# Autodesk Inventor assembly: brama kwadraty
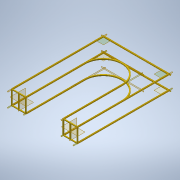
[picture p0: Inventor's stored thumbnail of the model, 180x180]
Saved by Autodesk Inventor 2021 (Build 250183000, 183)
## iProperties
Created: 2024-04-18
Part Number: brama kwadraty
Document SubType Name: Assembly
Designer: Michal
Author: Michal
## Documents named in this file (8)
- C:\Users\Michal\Documents\GitHub\PNW_PhotoBoothFrame_3D\brama kwadraty.iam
- C:\Users\Michal\Documents\GitHub\PNW_PhotoBoothFrame_3D\Lacznik prosty sruby.iam
- C:\Users\Michal\Documents\GitHub\PNW_PhotoBoothFrame_3D\Luk R1000.ipt
- C:\Users\Michal\Documents\GitHub\PNW_PhotoBoothFrame_3D\Stopa v3.iam
- C:\Users\Michal\Documents\GitHub\PNW_PhotoBoothFrame_3D\Naroznik v2.iam
- C:\Users\Michal\Documents\GitHub\PNW_PhotoBoothFrame_3D\Przedluzka L1680.ipt
- C:\Users\Michal\Documents\GitHub\PNW_PhotoBoothFrame_3D\Przedluzka L2400.ipt
- C:\Users\Michal\Documents\GitHub\PNW_PhotoBoothFrame_3D\Przedluzka L1360.ipt
## Components (22 placed, 7 different names)
1. Stopa v3:1 [sub-assembly] — Flush:1, Flush:2, Mate:40, Mate:64, Flush:3, Flush:5, Mate:88, Flush:10, Mate:89
2. Stopa v3:2 [sub-assembly] — Flush:1, Flush:2, Mate:41, Flush:4, Mate:67, Mate:68, Flush:13, Mate:101, Mate:102
3. Lacznik prosty sruby:1 [sub-assembly] — Mate:42, Mate:43, Mate:47, Mate:48, Mate:49
4. Przedluzka L1360:1 — Mate:40, Mate:42, Mate:43, Mate:64, Flush:3
5. Przedluzka L1360:2 — Mate:41, Mate:44, Mate:45, Mate:46, Flush:4
6. Lacznik prosty sruby:2 [sub-assembly] — Mate:44, Mate:45, Mate:46, Mate:50, Mate:51, Mate:52
7. Luk R1000:1 — Mate:47, Mate:48, Mate:49, Mate:50, Mate:51, Mate:52
8. Lacznik prosty sruby:3 [sub-assembly] — Mate:65, Mate:69
9. Przedluzka L1360:3 — Mate:67, Mate:68, Mate:69
10. Przedluzka L1360:4 — Flush:5
11. Lacznik prosty sruby:4 [sub-assembly] — Mate:66
12. Luk R1000:2 — Mate:65, Mate:66
13. Naroznik v2:1 [sub-assembly] — Mate:87
14. Przedluzka L2400:1 — Mate:87, Mate:88, Flush:10, Mate:89
15. Przedluzka L1680:1 — Flush:9, Mate:85, Mate:86
16. Naroznik v2:2 [sub-assembly] — Mate:83, Mate:84, Mate:85, Mate:86
17. Przedluzka L2400:2 — Mate:83, Mate:84, Flush:9
18. Naroznik v2:3 [sub-assembly] — Mate:100
19. Przedluzka L2400:3 — Mate:100, Flush:13, Mate:101, Mate:102
20. Przedluzka L1680:2 — Mate:98
21. Naroznik v2:4 [sub-assembly] — Mate:98, Mate:99
22. Przedluzka L2400:4 — Mate:99
## Relationships (63: Mate 52, Flush 11)
- Flush:1: Stopa v3:1 ↔ Stopa v3:2
- Flush:2: Stopa v3:1 ↔ Stopa v3:2
- Mate:40: Stopa v3:1 ↔ Przedluzka L1360:1
- Mate:41: Stopa v3:2 ↔ Przedluzka L1360:2
- Mate:42: Lacznik prosty sruby:1 ↔ Przedluzka L1360:1
- Mate:43: Lacznik prosty sruby:1 ↔ Przedluzka L1360:1
- Mate:44: Przedluzka L1360:2 ↔ Lacznik prosty sruby:2
- Mate:45: Przedluzka L1360:2 ↔ Lacznik prosty sruby:2
- Mate:46: Przedluzka L1360:2 ↔ Lacznik prosty sruby:2
- Mate:47: Lacznik prosty sruby:1 ↔ Luk R1000:1
- Mate:48: Lacznik prosty sruby:1 ↔ Luk R1000:1
- Mate:49: Lacznik prosty sruby:1 ↔ Luk R1000:1
- Mate:50: Lacznik prosty sruby:2 ↔ Luk R1000:1
- Mate:51: Lacznik prosty sruby:2 ↔ Luk R1000:1
- Mate:52: Lacznik prosty sruby:2 ↔ Luk R1000:1
- [Mate]: Lacznik prosty sruby:3 ↔ Przedluzka L1360:3
- [Mate]: Lacznik prosty sruby:3 ↔ Przedluzka L1360:3
- [Mate]: Przedluzka L1360:4 ↔ Lacznik prosty sruby:4
- [Mate]: Przedluzka L1360:4 ↔ Lacznik prosty sruby:4
- [Mate]: Przedluzka L1360:4 ↔ Lacznik prosty sruby:4
- [Mate]: Lacznik prosty sruby:3 ↔ Luk R1000:2
- [Mate]: Lacznik prosty sruby:3 ↔ Luk R1000:2
- [Mate]: Lacznik prosty sruby:4 ↔ Luk R1000:2
- [Mate]: Lacznik prosty sruby:4 ↔ Luk R1000:2
- Mate:64: Stopa v3:1 ↔ Przedluzka L1360:1
- Flush:3: Stopa v3:1 ↔ Przedluzka L1360:1
- Flush:4: Stopa v3:2 ↔ Przedluzka L1360:2
- Mate:65: Lacznik prosty sruby:3 ↔ Luk R1000:2
- Mate:66: Lacznik prosty sruby:4 ↔ Luk R1000:2
- Mate:67: Stopa v3:2 ↔ Przedluzka L1360:3
- Mate:68: Stopa v3:2 ↔ Przedluzka L1360:3
- Mate:69: Lacznik prosty sruby:3 ↔ Przedluzka L1360:3
- Flush:5: Stopa v3:1 ↔ Przedluzka L1360:4
- [Mate]: Naroznik v2:1 ↔ Przedluzka L2400:1
- [Mate]: Naroznik v2:1 ↔ Przedluzka L2400:1
- [Flush]: Naroznik v2:1 ↔ Przedluzka L1680:1
- [Mate]: Naroznik v2:1 ↔ Przedluzka L1680:1
- [Mate]: Naroznik v2:1 ↔ Przedluzka L1680:1
- [Mate]: Naroznik v2:2 ↔ Przedluzka L2400:2
- Mate:83: Naroznik v2:2 ↔ Przedluzka L2400:2
- Mate:84: Naroznik v2:2 ↔ Przedluzka L2400:2
- Flush:9: Przedluzka L1680:1 ↔ Przedluzka L2400:2
- Mate:85: Przedluzka L1680:1 ↔ Naroznik v2:2
- Mate:86: Przedluzka L1680:1 ↔ Naroznik v2:2
- Mate:87: Naroznik v2:1 ↔ Przedluzka L2400:1
- Mate:88: Stopa v3:1 ↔ Przedluzka L2400:1
- Flush:10: Stopa v3:1 ↔ Przedluzka L2400:1
- Mate:89: Stopa v3:1 ↔ Przedluzka L2400:1
- [Mate]: Naroznik v2:3 ↔ Przedluzka L2400:3
- [Mate]: Naroznik v2:3 ↔ Przedluzka L2400:3
- [Flush]: Naroznik v2:3 ↔ Przedluzka L1680:2
- [Mate]: Naroznik v2:3 ↔ Przedluzka L1680:2
- [Mate]: Naroznik v2:3 ↔ Przedluzka L1680:2
- [Mate]: Naroznik v2:4 ↔ Przedluzka L2400:4
- [Mate]: Naroznik v2:4 ↔ Przedluzka L2400:4
- [Flush]: Przedluzka L1680:2 ↔ Przedluzka L2400:4
- [Mate]: Przedluzka L1680:2 ↔ Naroznik v2:4
- Mate:98: Przedluzka L1680:2 ↔ Naroznik v2:4
- Mate:99: Naroznik v2:4 ↔ Przedluzka L2400:4
- Mate:100: Naroznik v2:3 ↔ Przedluzka L2400:3
- Flush:13: Stopa v3:2 ↔ Przedluzka L2400:3
- Mate:101: Stopa v3:2 ↔ Przedluzka L2400:3
- Mate:102: Stopa v3:2 ↔ Przedluzka L2400:3
## Named parameters: d92_d56 = 0 mm, d93_d57 = 0 mm, d94_d58 = 0 mm, d95_d59 = 0 mm, d96_d60 = 0 mm, d97_d86 = 0 mm, d98_d87 = 0 mm, d100_d89 = 0 mm, d102_d91 = 0 mm, d138_d129 = 0 mm, d139_d130 = 0 mm, d140_d131 = 0 mm, d143_d79 = 0 mm, d144_d80 = 0 mm, d145_d81 = 0 mm, d146_d85 = 0 mm, d147_d63 = 0 mm, d148_d68 = 0 mm
